# Autodesk Inventor assembly: BTSwitch
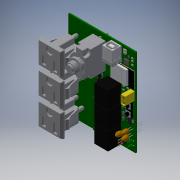
[picture p0: Inventor's stored thumbnail of the model, 180x180]
Saved by Autodesk Inventor 2019 (Build 230136000, 136)
## iProperties
Company: Open CASCADE
Created: 2019-01-21
Part Number: BTSwitch
Description: Open CASCADE Model
Document SubType Name: Assembly
Designer: Jorian Bruslind
Authority: Unknown
Sending System: Open CASCADE 6.5
Preprocessor: Open CASCADE STEP processor 6.5
Title: Open CASCADE Shape Model
Author: Author
## Documents named in this file (65)
- C:\Users\Jorian Bruslind\Documents\GitHub\SchoolWork\ECE341\Final Project\PCB Files\MK1.1\Bluetooth Switch\ExportSTEP\Inventor Version\BTSwitch.iam
- C:\Users\Jorian Bruslind\Documents\GitHub\SchoolWork\ECE341\Final Project\PCB Files\MK1.1\Bluetooth Switch\ExportSTEP\Inventor Version\Board.ipt
- C:\Users\Jorian Bruslind\Documents\GitHub\SchoolWork\ECE341\Final Project\PCB Files\MK1.1\Bluetooth Switch\ExportSTEP\Inventor Version\C8.iam
- C:\Users\Jorian Bruslind\Documents\GitHub\SchoolWork\ECE341\Final Project\PCB Files\MK1.1\Bluetooth Switch\ExportSTEP\Inventor Version\C7.iam
- C:\Users\Jorian Bruslind\Documents\GitHub\SchoolWork\ECE341\Final Project\PCB Files\MK1.1\Bluetooth Switch\ExportSTEP\Inventor Version\C6.iam
- C:\Users\Jorian Bruslind\Documents\GitHub\SchoolWork\ECE341\Final Project\PCB Files\MK1.1\Bluetooth Switch\ExportSTEP\Inventor Version\F1.iam
- C:\Users\Jorian Bruslind\Documents\GitHub\SchoolWork\ECE341\Final Project\PCB Files\MK1.1\Bluetooth Switch\ExportSTEP\Inventor Version\U5.iam
- C:\Users\Jorian Bruslind\Documents\GitHub\SchoolWork\ECE341\Final Project\PCB Files\MK1.1\Bluetooth Switch\ExportSTEP\Inventor Version\U2.iam
- C:\Users\Jorian Bruslind\Documents\GitHub\SchoolWork\ECE341\Final Project\PCB Files\MK1.1\Bluetooth Switch\ExportSTEP\Inventor Version\S2.iam
- C:\Users\Jorian Bruslind\Documents\GitHub\SchoolWork\ECE341\Final Project\PCB Files\MK1.1\Bluetooth Switch\ExportSTEP\Inventor Version\S1.iam
- C:\Users\Jorian Bruslind\Documents\GitHub\SchoolWork\ECE341\Final Project\PCB Files\MK1.1\Bluetooth Switch\ExportSTEP\Inventor Version\R21.iam
- C:\Users\Jorian Bruslind\Documents\GitHub\SchoolWork\ECE341\Final Project\PCB Files\MK1.1\Bluetooth Switch\ExportSTEP\Inventor Version\R20.iam
- C:\Users\Jorian Bruslind\Documents\GitHub\SchoolWork\ECE341\Final Project\PCB Files\MK1.1\Bluetooth Switch\ExportSTEP\Inventor Version\R19.iam
- C:\Users\Jorian Bruslind\Documents\GitHub\SchoolWork\ECE341\Final Project\PCB Files\MK1.1\Bluetooth Switch\ExportSTEP\Inventor Version\R18.iam
- C:\Users\Jorian Bruslind\Documents\GitHub\SchoolWork\ECE341\Final Project\PCB Files\MK1.1\Bluetooth Switch\ExportSTEP\Inventor Version\R17.iam
- C:\Users\Jorian Bruslind\Documents\GitHub\SchoolWork\ECE341\Final Project\PCB Files\MK1.1\Bluetooth Switch\ExportSTEP\Inventor Version\R16.iam
- C:\Users\Jorian Bruslind\Documents\GitHub\SchoolWork\ECE341\Final Project\PCB Files\MK1.1\Bluetooth Switch\ExportSTEP\Inventor Version\R15.iam
- C:\Users\Jorian Bruslind\Documents\GitHub\SchoolWork\ECE341\Final Project\PCB Files\MK1.1\Bluetooth Switch\ExportSTEP\Inventor Version\R14.iam
- C:\Users\Jorian Bruslind\Documents\GitHub\SchoolWork\ECE341\Final Project\PCB Files\MK1.1\Bluetooth Switch\ExportSTEP\Inventor Version\R13.iam
- C:\Users\Jorian Bruslind\Documents\GitHub\SchoolWork\ECE341\Final Project\PCB Files\MK1.1\Bluetooth Switch\ExportSTEP\Inventor Version\R12.iam
- C:\Users\Jorian Bruslind\Documents\GitHub\SchoolWork\ECE341\Final Project\PCB Files\MK1.1\Bluetooth Switch\ExportSTEP\Inventor Version\R11.iam
- C:\Users\Jorian Bruslind\Documents\GitHub\SchoolWork\ECE341\Final Project\PCB Files\MK1.1\Bluetooth Switch\ExportSTEP\Inventor Version\R10.iam
- C:\Users\Jorian Bruslind\Documents\GitHub\SchoolWork\ECE341\Final Project\PCB Files\MK1.1\Bluetooth Switch\ExportSTEP\Inventor Version\R9.iam
- C:\Users\Jorian Bruslind\Documents\GitHub\SchoolWork\ECE341\Final Project\PCB Files\MK1.1\Bluetooth Switch\ExportSTEP\Inventor Version\R8.iam
- C:\Users\Jorian Bruslind\Documents\GitHub\SchoolWork\ECE341\Final Project\PCB Files\MK1.1\Bluetooth Switch\ExportSTEP\Inventor Version\R7.iam
- C:\Users\Jorian Bruslind\Documents\GitHub\SchoolWork\ECE341\Final Project\PCB Files\MK1.1\Bluetooth Switch\ExportSTEP\Inventor Version\R6.iam
- C:\Users\Jorian Bruslind\Documents\GitHub\SchoolWork\ECE341\Final Project\PCB Files\MK1.1\Bluetooth Switch\ExportSTEP\Inventor Version\R5.iam
- C:\Users\Jorian Bruslind\Documents\GitHub\SchoolWork\ECE341\Final Project\PCB Files\MK1.1\Bluetooth Switch\ExportSTEP\Inventor Version\R4.iam
- C:\Users\Jorian Bruslind\Documents\GitHub\SchoolWork\ECE341\Final Project\PCB Files\MK1.1\Bluetooth Switch\ExportSTEP\Inventor Version\R3.iam
- C:\Users\Jorian Bruslind\Documents\GitHub\SchoolWork\ECE341\Final Project\PCB Files\MK1.1\Bluetooth Switch\ExportSTEP\Inventor Version\R2.iam
- C:\Users\Jorian Bruslind\Documents\GitHub\SchoolWork\ECE341\Final Project\PCB Files\MK1.1\Bluetooth Switch\ExportSTEP\Inventor Version\R1.iam
- C:\Users\Jorian Bruslind\Documents\GitHub\SchoolWork\ECE341\Final Project\PCB Files\MK1.1\Bluetooth Switch\ExportSTEP\Inventor Version\Q3.iam
- C:\Users\Jorian Bruslind\Documents\GitHub\SchoolWork\ECE341\Final Project\PCB Files\MK1.1\Bluetooth Switch\ExportSTEP\Inventor Version\Q2.iam
- C:\Users\Jorian Bruslind\Documents\GitHub\SchoolWork\ECE341\Final Project\PCB Files\MK1.1\Bluetooth Switch\ExportSTEP\Inventor Version\Q1.iam
- C:\Users\Jorian Bruslind\Documents\GitHub\SchoolWork\ECE341\Final Project\PCB Files\MK1.1\Bluetooth Switch\ExportSTEP\Inventor Version\N3.iam
- C:\Users\Jorian Bruslind\Documents\GitHub\SchoolWork\ECE341\Final Project\PCB Files\MK1.1\Bluetooth Switch\ExportSTEP\Inventor Version\N2.iam
- C:\Users\Jorian Bruslind\Documents\GitHub\SchoolWork\ECE341\Final Project\PCB Files\MK1.1\Bluetooth Switch\ExportSTEP\Inventor Version\N1.iam
- C:\Users\Jorian Bruslind\Documents\GitHub\SchoolWork\ECE341\Final Project\PCB Files\MK1.1\Bluetooth Switch\ExportSTEP\Inventor Version\K3.iam
- C:\Users\Jorian Bruslind\Documents\GitHub\SchoolWork\ECE341\Final Project\PCB Files\MK1.1\Bluetooth Switch\ExportSTEP\Inventor Version\J6.iam
- C:\Users\Jorian Bruslind\Documents\GitHub\SchoolWork\ECE341\Final Project\PCB Files\MK1.1\Bluetooth Switch\ExportSTEP\Inventor Version\J5.iam
- C:\Users\Jorian Bruslind\Documents\GitHub\SchoolWork\ECE341\Final Project\PCB Files\MK1.1\Bluetooth Switch\ExportSTEP\Inventor Version\J4.iam
- C:\Users\Jorian Bruslind\Documents\GitHub\SchoolWork\ECE341\Final Project\PCB Files\MK1.1\Bluetooth Switch\ExportSTEP\Inventor Version\J2.iam
- C:\Users\Jorian Bruslind\Documents\GitHub\SchoolWork\ECE341\Final Project\PCB Files\MK1.1\Bluetooth Switch\ExportSTEP\Inventor Version\J1.iam
- C:\Users\Jorian Bruslind\Documents\GitHub\SchoolWork\ECE341\Final Project\PCB Files\MK1.1\Bluetooth Switch\ExportSTEP\Inventor Version\D5.iam
- C:\Users\Jorian Bruslind\Documents\GitHub\SchoolWork\ECE341\Final Project\PCB Files\MK1.1\Bluetooth Switch\ExportSTEP\Inventor Version\D4.iam
- C:\Users\Jorian Bruslind\Documents\GitHub\SchoolWork\ECE341\Final Project\PCB Files\MK1.1\Bluetooth Switch\ExportSTEP\Inventor Version\D3.iam
- C:\Users\Jorian Bruslind\Documents\GitHub\SchoolWork\ECE341\Final Project\PCB Files\MK1.1\Bluetooth Switch\ExportSTEP\Inventor Version\D2.iam
- C:\Users\Jorian Bruslind\Documents\GitHub\SchoolWork\ECE341\Final Project\PCB Files\MK1.1\Bluetooth Switch\ExportSTEP\Inventor Version\D1.iam
- C:\Users\Jorian Bruslind\Documents\GitHub\SchoolWork\ECE341\Final Project\PCB Files\MK1.1\Bluetooth Switch\ExportSTEP\Inventor Version\C5.iam
- C:\Users\Jorian Bruslind\Documents\GitHub\SchoolWork\ECE341\Final Project\PCB Files\MK1.1\Bluetooth Switch\ExportSTEP\Inventor Version\C4.iam
- C:\Users\Jorian Bruslind\Documents\GitHub\SchoolWork\ECE341\Final Project\PCB Files\MK1.1\Bluetooth Switch\ExportSTEP\Inventor Version\C3.iam
- C:\Users\Jorian Bruslind\Documents\GitHub\SchoolWork\ECE341\Final Project\PCB Files\MK1.1\Bluetooth Switch\ExportSTEP\Inventor Version\C2.iam
- C:\Users\Jorian Bruslind\Documents\GitHub\SchoolWork\ECE341\Final Project\PCB Files\MK1.1\Bluetooth Switch\ExportSTEP\Inventor Version\C1.iam
- C:\Users\Jorian Bruslind\Documents\GitHub\SchoolWork\ECE341\Final Project\PCB Files\MK1.1\Bluetooth Switch\ExportSTEP\Inventor Version\ACS710_R_Sense.iam
- C:\Users\Jorian Bruslind\Documents\GitHub\SchoolWork\ECE341\Final Project\PCB Files\MK1.1\Bluetooth Switch\ExportSTEP\Inventor Version\5V.iam
- C:\Users\Jorian Bruslind\Documents\GitHub\SchoolWork\ECE341\Final Project\PCB Files\MK1.1\Bluetooth Switch\ExportSTEP\Inventor Version\3_3V.iam
- C:\Users\Jorian Bruslind\Documents\GitHub\SchoolWork\ECE341\Final Project\PCB Files\MK1.1\Bluetooth Switch\ExportSTEP\Inventor Version\K1.iam
- C:\Users\Jorian Bruslind\Documents\GitHub\SchoolWork\ECE341\Final Project\PCB Files\MK1.1\Bluetooth Switch\ExportSTEP\Inventor Version\K2.iam
- C:\Users\Jorian Bruslind\Documents\GitHub\SchoolWork\ECE341\Final Project\PCB Files\MK1.1\Bluetooth Switch\ExportSTEP\Inventor Version\M1.iam
- C:\Users\Jorian Bruslind\Documents\GitHub\SchoolWork\ECE341\Final Project\PCB Files\MK1.1\Bluetooth Switch\ExportSTEP\Inventor Version\U1.iam
- C:\Users\Jorian Bruslind\Documents\GitHub\SchoolWork\ECE341\Final Project\PCB Files\MK1.1\Bluetooth Switch\ExportSTEP\Inventor Version\U3.iam
- C:\Users\Jorian Bruslind\Documents\GitHub\SchoolWork\ECE341\Final Project\PCB Files\MK1.1\Bluetooth Switch\ExportSTEP\Inventor Version\U4.iam
- C:\Users\Jorian Bruslind\Documents\GitHub\SchoolWork\ECE341\Final Project\PCB Files\MK1.1\Bluetooth Switch\ExportSTEP\Inventor Version\R22.iam
- C:\Users\Jorian Bruslind\Documents\GitHub\SchoolWork\ECE341\Final Project\PCB Files\MK1.1\Bluetooth Switch\ExportSTEP\Inventor Version\R23.iam
- C:\Users\Jorian Bruslind\Documents\GitHub\SchoolWork\ECE341\Final Project\PCB Files\MK1.1\Bluetooth Switch\ExportSTEP\Inventor Version\J3.iam
## Components (64 placed, 64 different names)
1. 805 — Mate:1, Flush:1, Flush:2, Flush:3, Mate:3, Flush:4, Mate:4
2. 811 [sub-assembly]
3. 815 [sub-assembly]
4. 819 [sub-assembly]
5. 821 [sub-assembly]
6. 824 [sub-assembly]
7. 826 [sub-assembly]
8. 836 [sub-assembly]
9. 842 [sub-assembly]
10. 848 [sub-assembly]
11. 852 [sub-assembly]
12. 856 [sub-assembly]
13. 860 [sub-assembly]
14. 864 [sub-assembly]
15. 868 [sub-assembly]
16. 872 [sub-assembly]
17. 876 [sub-assembly]
18. 882 [sub-assembly]
19. 886 [sub-assembly]
20. 890 [sub-assembly]
21. 894 [sub-assembly]
22. 898 [sub-assembly]
23. 902 [sub-assembly]
24. 906 [sub-assembly]
25. 912 [sub-assembly]
26. 918 [sub-assembly]
27. 924 [sub-assembly]
28. 928 [sub-assembly]
29. 932 [sub-assembly]
30. 936 [sub-assembly]
31. 939 [sub-assembly]
32. 941 [sub-assembly]
33. 943 [sub-assembly]
34. 957 [sub-assembly]
35. 965 [sub-assembly]
36. 973 [sub-assembly]
37. 975 [sub-assembly]
38. 977 [sub-assembly] — Mate:1, Flush:1, Flush:2, Mate:2
39. 979 [sub-assembly] — Mate:2, Flush:3, Mate:3, Mate:5
40. 981 [sub-assembly] — Flush:4, Mate:4, Mate:5
41. 987 [sub-assembly]
42. 989 [sub-assembly]
43. 992 [sub-assembly]
44. 994 [sub-assembly]
45. 996 [sub-assembly]
46. 998 [sub-assembly]
47. 1000 [sub-assembly]
48. 1004 [sub-assembly]
49. 1008 [sub-assembly]
50. 1013 [sub-assembly]
51. 1015 [sub-assembly]
52. 1017 [sub-assembly]
53. 1023 [sub-assembly]
54. 1034 [sub-assembly]
55. 1042 [sub-assembly]
56. 1044 [sub-assembly]
57. 1046 [sub-assembly]
58. 1048 [sub-assembly]
59. 1050 [sub-assembly]
60. 1052 [sub-assembly]
61. 1055 [sub-assembly]
62. 1059 [sub-assembly]
63. 1063 [sub-assembly]
64. 1072 [sub-assembly]
## Relationships (9: Mate 5, Flush 4)
- Mate:1 (12 mm): 805 ↔ 977
- Flush:1 (6 mm): 805 ↔ 977
- Flush:2 (7.5 mm): 805 ↔ 977
- Mate:2 (3 mm): 977 ↔ 979
- Flush:3 (6 mm): 805 ↔ 979
- Mate:3 (12 mm): 805 ↔ 979
- Flush:4 (6 mm): 805 ↔ 981
- Mate:4 (12 mm): 805 ↔ 981
- Mate:5 (3 mm): 979 ↔ 981
